# Autodesk Inventor assembly: ASY MSC 100 CONE
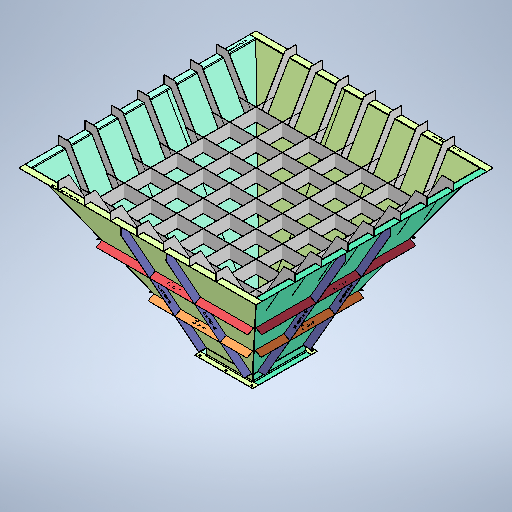
[picture p0: Inventor's stored thumbnail of the model, 512x512]
Saved by Autodesk Inventor 2025 (Build 290162010, 162A)
## iProperties
Created: 2024-05-19
Part Number: ASY MSC 100 CONE
Document SubType Name: Assembly
Designer: admin
Mass: 170206 g
Surface Area: 120081 cm^2
Volume: 21304.1 cm^3
Density: 7.98935 g/cm^3
Stock Number: ASY МОО 100 конус
Author: admin
## Documents named in this file (14)
- C:\Users\pokla\Documents\Inventor\NDM-VOS_powder_hopper\Workspaces\Workspace\Cone\ASY MSC 100 cone.iam
- C:\Users\pokla\Documents\Inventor\NDM-VOS_powder_hopper\Workspaces\Workspace\Cone\MSC 114 cone IN right board.ipt
- C:\Users\pokla\Documents\Inventor\NDM-VOS_powder_hopper\Workspaces\Workspace\Cone\MSC 113 cone IN left board.ipt
- C:\Users\pokla\Documents\Inventor\NDM-VOS_powder_hopper\Workspaces\Workspace\Cone\MSC 112 cone IN back.ipt
- C:\Users\pokla\Documents\Inventor\NDM-VOS_powder_hopper\Workspaces\Workspace\Cone\MSC DIM 001 cone sketch.ipt
- C:\Users\pokla\Documents\Inventor\NDM-VOS_powder_hopper\Workspaces\Workspace\Cone\MSC 115 cone IN bow.ipt
- C:\Users\pokla\Documents\Inventor\NDM-VOS_powder_hopper\Workspaces\Workspace\Cone\MSC 110 stringer cone.ipt
- C:\Users\pokla\Documents\Inventor\NDM-VOS_powder_hopper\Workspaces\Workspace\Cone\MSC 106 rib cone.ipt
- C:\Users\pokla\Documents\Inventor\NDM-VOS_powder_hopper\Workspaces\Workspace\Cone\MSC 107 rib cone.ipt
- C:\Users\pokla\Documents\Inventor\NDM-VOS_powder_hopper\Workspaces\Workspace\Cone\MSC 108 rib cone.ipt
- C:\Users\pokla\Documents\Inventor\NDM-VOS_powder_hopper\Workspaces\Workspace\Cone\MSC 109 rib cone.ipt
- C:\Users\pokla\Documents\Inventor\NDM-VOS_powder_hopper\NDM-VOS dummy2.ipt
- C:\Users\pokla\Documents\Inventor\NDM-VOS_powder_hopper\Workspaces\Workspace\Cone\MSC 201 GRID.ipt
- C:\Users\pokla\Documents\Inventor\NDM-VOS_powder_hopper\Workspaces\Workspace\Cone\MSC 202 GRID CORNER.ipt
## Components (65 placed, 19 different names)
1. NDM-VOS dummy2:1 — Mate:73, Mate:74, Flush:19
2. MSC DIM 001 CONE SKETCH:1 — Flush:8, Flush:9, Mate:1
3. MSC 112 CONE IN BACK:1 — Flush:6, Flush:10, Mate:2
4. MSC 114 CONE IN RIGHT BOARD:1 — Flush:13, Flush:15, Flush:18, Mate:79, Mate:81, Mate:82
5. MSC 113 CONE IN LEFT BOARD:1 — Mate:4, Flush:14, Mate:5
6. MSC 115 CONE IN BOW:1 — Mate:6, Flush:16, Flush:17
7. MSC 115 cone IN bow:2 — Mate:75, Flush:20, Flush:21, Mate:76, Mate:78, Mate:85
8. MSC 106 RIB CONE:1 — Rigid:7, Rigid:8, Mate:77
9. MSC 109 RIB CONE:1 — Rigid:6
10. MSC 110 STRINGER CONE:4 — Rigid:4, Rigid:6, Mate:79, Mate:81
11. MSC 108 RIB CONE:1 — Rigid:4, Rigid:5, Mate:80
12. MSC 110 STRINGER CONE:3 — Rigid:5
13. MSC 110 STRINGER CONE:2 — Rigid:8, Rigid:9
14. MSC 107 RIB CONE:1 — Rigid:9
15. MSC 110 STRINGER CONE:1 — Rigid:7, Mate:76, Mate:78
16. MSC 106 rib cone:2
17. MSC 109 rib cone:2
18. MSC 110 stringer cone:6
19. MSC 108 rib cone:2
20. MSC 110 stringer cone:7
21. MSC 110 stringer cone:8
22. MSC 107 rib cone:2
23. MSC 110 stringer cone:9
24. MSC 202 GRID CORNER:4 — Mate:85
25. MSC 201 GRID:2 — Mate:84, Mate:86
26. MSC 202 GRID CORNER:3
27. MSC 202 GRID CORNER:5
28. MSC 201 GRID:3
29. MSC 202 GRID CORNER:6
30. MSC 202 GRID CORNER:7
31. MSC 201 GRID:4
32. MSC 202 GRID CORNER:8
33. MSC 202 GRID CORNER:9
34. MSC 201 GRID:5
35. MSC 202 GRID CORNER:10
36. MSC 202 GRID CORNER:11
37. MSC 201 GRID:6
38. MSC 202 GRID CORNER:12
39. MSC 202 GRID CORNER:13
40. MSC 201 GRID:7
41. MSC 202 GRID CORNER:14
42. MSC 202 GRID CORNER:15
43. MSC 201 GRID:8
44. MSC 202 GRID CORNER:16
45. MSC 202 GRID CORNER:2 — Rigid:11
46. MSC 201 GRID:1 — Rigid:10, Rigid:11, Flush:22, Mate:83
47. MSC 202 GRID CORNER:1 — Rigid:10, Mate:82
48. MSC 202 GRID CORNER:19
49. MSC 201 GRID:10
50. MSC 202 GRID CORNER:20
51. MSC 202 GRID CORNER:21
52. MSC 201 GRID:11
53. MSC 202 GRID CORNER:22
54. MSC 202 GRID CORNER:23
55. MSC 201 GRID:12
56. MSC 202 GRID CORNER:24
57. MSC 202 GRID CORNER:25
58. MSC 201 GRID:13
59. MSC 202 GRID CORNER:26
60. MSC 202 GRID CORNER:27
61. MSC 201 GRID:14
62. MSC 202 GRID CORNER:28
63. MSC 202 GRID CORNER:29
64. MSC 201 GRID:15
65. MSC 202 GRID CORNER:30
## Component patterns: (2 elements, first: MSC 106 RIB CONE:1 + MSC 109 RIB CONE:1 + MSC 110 STRINGER CONE:4 + MSC 108 RIB CONE:1 + MSC 110 STRINGER CONE:3 + MSC 110 STRINGER CONE:2 + MSC 107 RIB CONE:1 + MSC 110 STRINGER CONE:1), (7 elements, first: MSC 202 GRID CORNER:4 + MSC 201 GRID:2 + MSC 202 GRID CORNER:3), (7 elements, first: MSC 202 GRID CORNER:2 + MSC 201 GRID:1 + MSC 202 GRID CORNER:1)
## Relationships (43: Mate 19, Flush 14, WeldJoint 10)
- Flush:6: MSC 112 CONE IN BACK:1
- Flush:8: MSC DIM 001 CONE SKETCH:1
- Flush:9: MSC DIM 001 CONE SKETCH:1
- Mate:1: MSC DIM 001 CONE SKETCH:1
- Flush:10: MSC 112 CONE IN BACK:1
- Mate:2: MSC 112 CONE IN BACK:1
- Flush:13: MSC 114 CONE IN RIGHT BOARD:1
- Mate:4: MSC 113 CONE IN LEFT BOARD:1
- Flush:14: MSC 113 CONE IN LEFT BOARD:1
- Mate:5: MSC 113 CONE IN LEFT BOARD:1
- Flush:15: MSC 114 CONE IN RIGHT BOARD:1
- Mate:6: MSC 115 CONE IN BOW:1
- Flush:16: MSC 115 CONE IN BOW:1
- Flush:17: MSC 115 CONE IN BOW:1
- Rigid:4 [WeldJoint] (2 mm): MSC 110 STRINGER CONE:4 ↔ MSC 108 RIB CONE:1
- Rigid:5 [WeldJoint] (2 mm): MSC 108 RIB CONE:1 ↔ MSC 110 STRINGER CONE:3
- Rigid:6 [WeldJoint] (2 mm): MSC 109 RIB CONE:1 ↔ MSC 110 STRINGER CONE:4
- Rigid:7 [WeldJoint] (2 mm): MSC 106 RIB CONE:1 ↔ MSC 110 STRINGER CONE:1
- Rigid:8 [WeldJoint] (2 mm): MSC 106 RIB CONE:1 ↔ MSC 110 STRINGER CONE:2
- Rigid:9 [WeldJoint] (2 mm): MSC 110 STRINGER CONE:2 ↔ MSC 107 RIB CONE:1
- Flush:18: MSC 114 CONE IN RIGHT BOARD:1
- Mate:73: NDM-VOS dummy2:1
- Mate:74: NDM-VOS dummy2:1
- Flush:19: NDM-VOS dummy2:1
- Mate:75: MSC 115 cone IN bow:2
- Flush:20: MSC 115 cone IN bow:2
- Flush:21: MSC 115 cone IN bow:2
- Mate:76: MSC 115 cone IN bow:2 ↔ MSC 110 STRINGER CONE:1
- Mate:77: MSC 106 RIB CONE:1
- Mate:78 (2 mm): MSC 115 cone IN bow:2 ↔ MSC 110 STRINGER CONE:1
- Mate:79: MSC 114 CONE IN RIGHT BOARD:1 ↔ MSC 110 STRINGER CONE:4
- Mate:80: MSC 108 RIB CONE:1
- Mate:81 (4 mm): MSC 114 CONE IN RIGHT BOARD:1 ↔ MSC 110 STRINGER CONE:4
- Rigid:10 [WeldJoint]: MSC 201 GRID:1 ↔ MSC 202 GRID CORNER:1
- Rigid:11 [WeldJoint]: MSC 202 GRID CORNER:2 ↔ MSC 201 GRID:1
- [WeldJoint]: MSC 201 GRID:2 ↔ MSC 202 GRID CORNER:3
- [WeldJoint]: MSC 202 GRID CORNER:4 ↔ MSC 201 GRID:2
- Flush:22: MSC 201 GRID:1
- Mate:82: MSC 114 CONE IN RIGHT BOARD:1 ↔ MSC 202 GRID CORNER:1
- Mate:83: MSC 201 GRID:1
- Mate:84: MSC 201 GRID:2
- Mate:85: MSC 115 cone IN bow:2 ↔ MSC 202 GRID CORNER:4
- Mate:86: MSC 201 GRID:2
## Named parameters: Конус_Базовая_Высота = 1170 mm, Конус_отступ_от_пола = 0 mm, d200_d198 = 0 mm, d201_d199 = 0 mm
